# Autodesk Inventor assembly: vidasız montaj
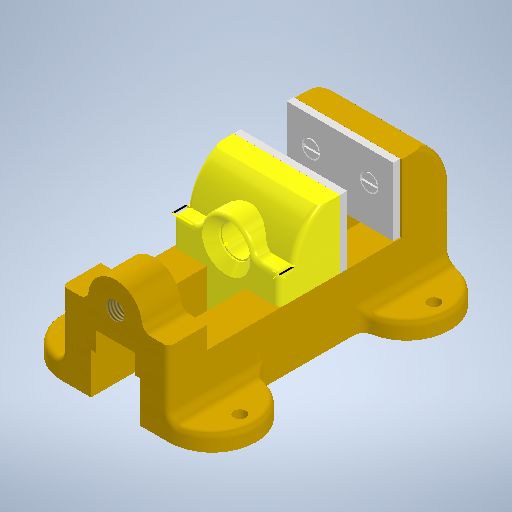
[picture p0: Inventor's stored thumbnail of the model, 512x512]
Saved by Autodesk Inventor 2025.4 (Build 294407000, 407)
## iProperties
Created: 2026-06-22
Part Number: vidasız montaj
Document SubType Name: Assembly
Designer: win10
Author: win10
## Documents named in this file (5)
- C:\Users\win10\Desktop\cad-final-projesi\vidasız montaj.iam
- C:\Users\win10\Desktop\cad-final-projesi\alt_plaka.ipt
- C:\Users\win10\Desktop\cad-final-projesi\haraketli_palaka.ipt
- C:\Users\win10\Desktop\cad-final-projesi\plaka.ipt
- C:\Users\win10\Documents\Inventor\Content Center Files\R2025\en-US\AS 1427(03)\AS 1427 - M6 x 16(1).ipt
## Components (8 placed, 4 different names)
1. alt_plaka:1 — Mate:1, Mate:2, Insert:1, Insert:2
2. plaka:1 — Insert:1, Insert:2, Insert:7, Insert:8
3. haraketli_palaka:1 — Mate:1, Mate:2, Insert:9, Insert:10
4. AS 1427 - Metric M6 x 16:1 — Insert:8
5. AS 1427 - Metric M6 x 16:2 — Insert:7
6. AS 1427 - Metric M6 x 16:3 — Insert:11
7. AS 1427 - Metric M6 x 16:4 — Insert:12
8. plaka:2 — Insert:9, Insert:10, Insert:11, Insert:12
## Relationships (10: Insert 8, Mate 2)
- Mate:1: alt_plaka:1 ↔ haraketli_palaka:1
- Mate:2: alt_plaka:1 ↔ haraketli_palaka:1
- Insert:1: alt_plaka:1 ↔ plaka:1
- Insert:2: alt_plaka:1 ↔ plaka:1
- Insert:7: plaka:1 ↔ AS 1427 - Metric M6 x 16:2
- Insert:8: plaka:1 ↔ AS 1427 - Metric M6 x 16:1
- Insert:9: haraketli_palaka:1 ↔ plaka:2
- Insert:10: haraketli_palaka:1 ↔ plaka:2
- Insert:11: AS 1427 - Metric M6 x 16:3 ↔ plaka:2
- Insert:12: AS 1427 - Metric M6 x 16:4 ↔ plaka:2
